# Autodesk Inventor assembly: Shock Strut
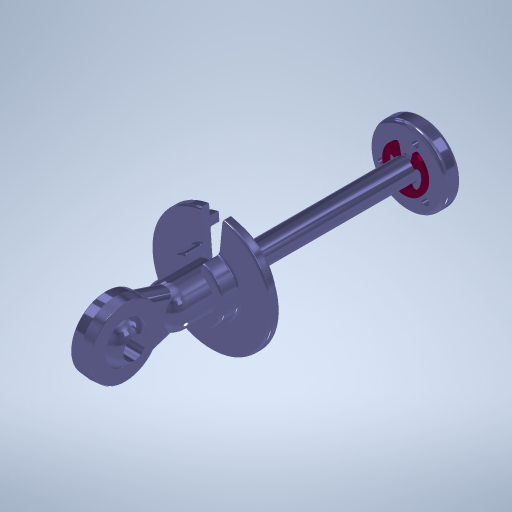
[picture p0: Inventor's stored thumbnail of the model, 512x512]
Saved by Autodesk Inventor 2023.1 (Build 271208000, 208)
## iProperties
Created: 2019-12-01
Part Number: Shock Strut
Document SubType Name: Assembly
Designer: Jopa
Author: Jopa
## Documents named in this file (6)
- C:\Users\Arzum Naz Doğaner\OneDrive\Masaüstü\HUDSON süspansiyon\Shock Strut.iam
- C:\Users\Arzum Naz Doğaner\OneDrive\Masaüstü\HUDSON süspansiyon\Shock Shaft.ipt
- C:\Users\Arzum Naz Doğaner\OneDrive\Masaüstü\HUDSON süspansiyon\Piston of Suspension.ipt
- C:\Users\Arzum Naz Doğaner\OneDrive\Masaüstü\HUDSON süspansiyon\E-Clip.ipt
- C:\Users\Arzum Naz Doğaner\OneDrive\Masaüstü\HUDSON süspansiyon\Ball End.iam
- C:\Users\Arzum Naz Doğaner\OneDrive\Masaüstü\HUDSON süspansiyon\Spring Cup.ipt
## Components (6 placed, 5 different names)
1. Shock Shaft:1 — Mate:1, Flush:1, Mate:6, Mate:7, Mate:9
2. Piston of Suspension:1 — Mate:1, Mate:2, Mate:3, Mate:4, Mate:5, Flush:1
3. E-Clip:1 — Mate:4, Mate:5
4. E-Clip:2 — Mate:2, Mate:3
5. Ball End:1 [sub-assembly] — Mate:6, Mate:7, Mate:8
6. Spring Cup:1 — Mate:8, Mate:9
## Relationships (10: Mate 9, Flush 1)
- Mate:1: Shock Shaft:1 ↔ Piston of Suspension:1
- Mate:2: Piston of Suspension:1 ↔ E-Clip:2
- Mate:3: Piston of Suspension:1 ↔ E-Clip:2
- Mate:4: Piston of Suspension:1 ↔ E-Clip:1
- Mate:5: Piston of Suspension:1 ↔ E-Clip:1
- Flush:1: Shock Shaft:1 ↔ Piston of Suspension:1
- Mate:6: Shock Shaft:1 ↔ Ball End:1
- Mate:7: Shock Shaft:1 ↔ Ball End:1
- Mate:8: Ball End:1 ↔ Spring Cup:1
- Mate:9: Shock Shaft:1 ↔ Spring Cup:1
